# Autodesk Inventor assembly: Assembly2
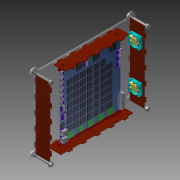
[picture p0: Inventor's stored thumbnail of the model, 180x180]
Saved by Autodesk Inventor 2015 (Build 190159000, 159)
## iProperties
Created: 2014-08-07
Part Number: Assembly2
Document SubType Name: Assembly
Designer: Patrick Camilleri
Author: Patrick Camilleri
## Documents named in this file (8)
- C:\Users\Patrick Camilleri\CAD\Test Box\Assembly2.iam
- C:\Users\Patrick Camilleri\CAD\Test Box\BasePlate2.ipt
- C:\Users\Patrick Camilleri\CAD\Test Box\SidePanel_GuideRail.iam
- C:\Users\Patrick Camilleri\CAD\Test Box\SidePanel_GuideRail_MIR1.iam
- C:\Users\Patrick Camilleri\CAD\Spin5 Board\Spin5 Inventor Simple 2\Imported Components\spin5v1_simple_2\spin5v1_simple_2.iam
- C:\Users\Patrick Camilleri\CAD\Test Box\Panel4.ipt
- C:\Users\Patrick Camilleri\CAD\Test Box\SidePanelFans2.iam
- C:\Users\Patrick Camilleri\CAD\Test Box\Bolt1.iam
## Components (11 placed, 7 different names)
1. BasePlate2:1 — Rigid:1, Rigid:3, Rigid:4
2. SidePanel_GuideRail:1 [sub-assembly]
3. SidePanel_GuideRail_MIR1:1 [sub-assembly] — Rigid:1, Rigid:2
4. spin5v1_simple_2:1 [sub-assembly] — Rigid:2
5. Panel4:1 — Rigid:3
6. SidePanelFans2:1 [sub-assembly] — Rigid:4, Rigid:5
7. BasePlate2:2 — Rigid:5, Rigid:9, Rigid:10, Rigid:11
8. Bolt1:1 [sub-assembly]
9. Bolt1:2 [sub-assembly] — Rigid:11
10. Bolt1:3 [sub-assembly] — Rigid:10
11. Bolt1:4 [sub-assembly] — Rigid:9
## Relationships (10: WeldJoint 10)
- Rigid:1 [WeldJoint]: BasePlate2:1 ↔ SidePanel_GuideRail_MIR1:1
- Rigid:2 [WeldJoint]: SidePanel_GuideRail_MIR1:1 ↔ spin5v1_simple_2:1
- Rigid:3 [WeldJoint]: BasePlate2:1 ↔ Panel4:1
- Rigid:4 [WeldJoint]: BasePlate2:1 ↔ SidePanelFans2:1
- Rigid:5 [WeldJoint]: SidePanelFans2:1 ↔ BasePlate2:2
- [WeldJoint]: BasePlate2:2 ↔ Bolt1:1
- [WeldJoint]: BasePlate2:1 ↔ Bolt1:1
- Rigid:9 [WeldJoint]: BasePlate2:2 ↔ Bolt1:4
- Rigid:10 [WeldJoint]: BasePlate2:2 ↔ Bolt1:3
- Rigid:11 [WeldJoint]: BasePlate2:2 ↔ Bolt1:2
